# Autodesk Inventor assembly: BodyV4_MIR_Left
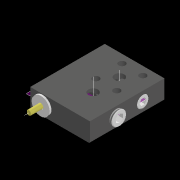
[picture p0: Inventor's stored thumbnail of the model, 180x180]
Saved by Autodesk Inventor 2021 (Build 250183000, 183)
## iProperties
Created: 2024-03-17
Part Number: BodyV4_MIR_Left
Document SubType Name: Assembly
Designer: top10
Author: top10
## Documents named in this file (5)
- D:\Files\Graduation Project\V4_manfoulid\Workspaces\Workspace\MIR_Left\BodyV4_MIR_Left.iam
- D:\Files\Graduation Project\V4_manfoulid\Workspaces\Workspace\MIR_Left\Val_BodV4_MIR_Left.ipt
- D:\Files\Graduation Project\V4_manfoulid\Workspaces\Workspace\R_nozzle\MIR_Left\rotarynozzle_MIR_Left.iam
- D:\Files\Graduation Project\V4_manfoulid\Workspaces\Workspace\MIR_Left\M10_HEX_MIR_Left.ipt
- D:\Files\Graduation Project\V4_manfoulid\Workspaces\Workspace\MIR_Left\M12_HEX_MIR_Left.ipt
## Components (4 placed, 4 different names)
1. Val_BodV4_MIR_Left:1 — Flush:3, Flush:2, Flush:1, Mate:1, Mate:3, Mate:2, Flush:4, Mate:7, Mate:8
2. rotarynozzle_MIR_Left:1 [sub-assembly] — Mate:1, Mate:3, Mate:2
3. M10_HEX_MIR_Left:1 — Flush:4, Mate:7
4. M12_HEX_MIR_Left:1 — Mate:8
## Relationships (9: Mate 5, Flush 4)
- Flush:3: Val_BodV4_MIR_Left:1
- Flush:2: Val_BodV4_MIR_Left:1
- Flush:1: Val_BodV4_MIR_Left:1
- Mate:1 (-20 mm): Val_BodV4_MIR_Left:1 ↔ rotarynozzle_MIR_Left:1
- Mate:3: Val_BodV4_MIR_Left:1 ↔ rotarynozzle_MIR_Left:1
- Mate:2: Val_BodV4_MIR_Left:1 ↔ rotarynozzle_MIR_Left:1
- Flush:4: Val_BodV4_MIR_Left:1 ↔ M10_HEX_MIR_Left:1
- Mate:7: Val_BodV4_MIR_Left:1 ↔ M10_HEX_MIR_Left:1
- Mate:8: Val_BodV4_MIR_Left:1 ↔ M12_HEX_MIR_Left:1
